# Autodesk Inventor assembly: drive
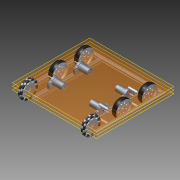
[picture p0: Inventor's stored thumbnail of the model, 180x180]
Saved by Autodesk Inventor 2013 (Build 170138000, 138)
## iProperties
Created: 2013-09-22
Part Number: drive
Document SubType Name: Assembly
Designer: Family Room
Mass: 858.54 g
Surface Area: 8628.43 cm^2
Volume: 788.69 cm^3
Density: 1.08856 g/cm^3
Author: Family Room
## Documents named in this file (12)
- C:\Users\cobrooks\Documents\GitHub\2013-2014_BlockParty\CAD\Drive\WIMP_mk2\drive.iam
- C:\Users\cobrooks\Documents\GitHub\2013-2014_BlockParty\CAD\Drive\Final Drive Complete\Frame Layer open.iam
- C:\Users\Family Room\Documents\Inventor\Content Center Files\R2011\en-US\ANSI B18.3(13)\ANSI B18.3 - 1_4-28 UNF - 1(22).ipt
- C:\Users\cobrooks\Documents\GitHub\2013-2014_BlockParty\CAD\Drive\Final Drive Complete\Tetrix Wheel 4 in omni.ipt
- C:\Users\cobrooks\Documents\GitHub\2013-2014_BlockParty\CAD\Drive\Final Drive Complete\Tetrix wheel 4 in.ipt
- C:\Users\cobrooks\Documents\GitHub\2013-2014_BlockParty\CAD\Drive\Final Drive Complete\pvc holder.ipt
- C:\Users\rihoobler\Documents\Inventor\tetrix_739091_2012.ipt
- U:\Imported Components\tetrix_739088_2012\tetrix_739088_2012.ipt
- U:\Imported Components\tetrix_739165_2012\tetrix_739165_2012.ipt
- U:\Imported Components\tetrix_739172_2012\tetrix_739172_2012.iam
- C:\Users\cobrooks\Documents\GitHub\2013-2014_BlockParty\CAD\Drive\Final Drive Complete\Motor Mount.ipt
- C:\Users\cobrooks\Documents\GitHub\2013-2014_BlockParty\CAD\Drive\Final Drive Complete\Motor.iam
## Components (61 placed, 11 different names)
1. Frame Layer open:1 [sub-assembly] — Insert:4, Insert:5, Insert:6, Mate:37, Mate:38, Flush:44, Mate:72, Flush:50, Mate:74, Flush:51, Mate:76, Flush:52, Flush:53, Mate:77, Flush:60
2. Spline Socket Head Cap Screw - Inch 1/4-28 UNF - 1:1
3. Spline Socket Head Cap Screw - Inch 1/4-28 UNF - 1:2
4. Spline Socket Head Cap Screw - Inch 1/4-28 UNF - 1:3
5. Spline Socket Head Cap Screw - Inch 1/4-28 UNF - 1:4 — Insert:4
6. Spline Socket Head Cap Screw - Inch 1/4-28 UNF - 1:5 — Insert:5
7. Spline Socket Head Cap Screw - Inch 1/4-28 UNF - 1:6 — Insert:6
8. Tetrix Wheel 4 in omni:1 — Mate:40, Mate:42, Mate:43, Flush:36, Insert:19
9. Tetrix Wheel 4 in omni:2 — Mate:41, Mate:44, Mate:45, Insert:24
10. Tetrix wheel 4 in:1 — Flush:34, Insert:26
11. Tetrix wheel 4 in:2 — Flush:34, Flush:35, Insert:25
12. Tetrix wheel 4 in:3 — Flush:36, Flush:37, Insert:21
13. Tetrix wheel 4 in:4 — Flush:37, Insert:22
14. pvc holder:1
15. pvc holder:2
16. pvc holder:3 — Mate:38
17. pvc holder:4 — Mate:37
18. Tetrix Wheel 4 in omni:3 — Mate:40, Mate:42, Mate:43, Insert:20
19. Tetrix Wheel 4 in omni:4 — Mate:41, Mate:44, Mate:45, Flush:35, Insert:27
20. tetrix_739091_2012:1 — Mate:50
21. tetrix_739091_2012:2 — Mate:61
22. tetrix_739091_2012:3
23. tetrix_739091_2012:4 — Mate:51
24. tetrix_739091_2012:5 — Mate:52
25. tetrix_739091_2012:6
26. tetrix_739091_2012:7
27. tetrix_739091_2012:8 — Flush:38, Mate:53
28. tetrix_739091_2012:9
29. tetrix_739091_2012:10 — Flush:38, Flush:39, Mate:54
30. tetrix_739091_2012:11
31. tetrix_739091_2012:12 — Flush:39, Mate:55, Mate:67
32. tetrix_739088_2012:1 — Mate:50
33. tetrix_739088_2012:2 — Mate:51, Flush:44, Flush:45, Mate:60
34. tetrix_739088_2012:3 — Mate:52, Flush:45, Mate:65
35. tetrix_739088_2012:4 — Mate:53
36. tetrix_739088_2012:5 — Mate:54, Mate:68, Mate:69
37. tetrix_739088_2012:6 — Mate:55, Mate:71
38. tetrix_739165_2012:1 — Insert:19, Flush:46
39. tetrix_739165_2012:2 — Mate:63, Mate:64, Mate:66, Flush:47
40. tetrix_739165_2012:3 — Mate:60, Flush:46, Mate:63, Mate:64, Insert:23
41. tetrix_739165_2012:4 — Mate:68, Flush:48, Insert:28
42. tetrix_739165_2012:5 — Insert:27, Flush:48
43. tetrix_739165_2012:6 — Mate:65, Flush:47
44. tetrix_739172_2012:1 [sub-assembly] — Insert:20, Mate:61
45. tetrix_739172_2012:2 [sub-assembly] — Insert:21
46. tetrix_739172_2012:3 [sub-assembly] — Insert:22
47. tetrix_739172_2012:4 [sub-assembly] — Insert:23, Mate:66
48. tetrix_739172_2012:5 [sub-assembly] — Insert:26, Mate:67
49. tetrix_739172_2012:6 [sub-assembly] — Insert:25
50. tetrix_739172_2012:7 [sub-assembly] — Insert:24
51. tetrix_739172_2012:8 [sub-assembly] — Insert:28, Mate:70
52. tetrix_739165_2012:7 — Mate:71, Flush:49
53. tetrix_739165_2012:8 — Mate:69, Mate:70, Flush:49
54. Motor Mount:1 — Mate:72, Flush:50, Flush:55, Mate:78, Flush:57
55. Motor Mount:2 — Mate:74, Flush:51, Flush:54, Mate:79, Flush:56
56. Motor Mount:3 — Mate:76, Flush:52, Flush:55, Mate:80, Flush:58
57. Motor Mount:4 — Flush:53, Mate:77, Flush:54, Mate:81, Flush:59
58. Motor:1 [sub-assembly] — Mate:78, Flush:57
59. Motor:2 [sub-assembly] — Mate:79, Flush:56
60. Motor:3 [sub-assembly] — Mate:80, Flush:58
61. Motor:4 [sub-assembly] — Mate:81, Flush:59
## Relationships (71: Mate 33, Flush 25, Insert 13)
- Insert:4: Frame Layer open:1 ↔ Spline Socket Head Cap Screw - Inch 1/4-28 UNF - 1:4
- Insert:5: Frame Layer open:1 ↔ Spline Socket Head Cap Screw - Inch 1/4-28 UNF - 1:5
- Insert:6: Frame Layer open:1 ↔ Spline Socket Head Cap Screw - Inch 1/4-28 UNF - 1:6
- Mate:37: Frame Layer open:1 ↔ pvc holder:4
- Mate:38: Frame Layer open:1 ↔ pvc holder:3
- Mate:40: Tetrix Wheel 4 in omni:1 ↔ Tetrix Wheel 4 in omni:3
- Mate:41: Tetrix Wheel 4 in omni:2 ↔ Tetrix Wheel 4 in omni:4
- Mate:42: Tetrix Wheel 4 in omni:1 ↔ Tetrix Wheel 4 in omni:3
- Mate:43: Tetrix Wheel 4 in omni:1 ↔ Tetrix Wheel 4 in omni:3
- Mate:44: Tetrix Wheel 4 in omni:2 ↔ Tetrix Wheel 4 in omni:4
- Mate:45: Tetrix Wheel 4 in omni:2 ↔ Tetrix Wheel 4 in omni:4
- Flush:34: Tetrix wheel 4 in:1 ↔ Tetrix wheel 4 in:2
- Flush:35: Tetrix wheel 4 in:2 ↔ Tetrix Wheel 4 in omni:4
- Flush:36: Tetrix Wheel 4 in omni:1 ↔ Tetrix wheel 4 in:3
- Flush:37: Tetrix wheel 4 in:3 ↔ Tetrix wheel 4 in:4
- Flush:38: tetrix_739091_2012:8 ↔ tetrix_739091_2012:10
- Flush:39: tetrix_739091_2012:10 ↔ tetrix_739091_2012:12
- Mate:50: tetrix_739091_2012:1 ↔ tetrix_739088_2012:1
- Mate:51: tetrix_739091_2012:4 ↔ tetrix_739088_2012:2
- Mate:52: tetrix_739091_2012:5 ↔ tetrix_739088_2012:3
- Mate:53: tetrix_739091_2012:8 ↔ tetrix_739088_2012:4
- Mate:54: tetrix_739091_2012:10 ↔ tetrix_739088_2012:5
- Mate:55: tetrix_739091_2012:12 ↔ tetrix_739088_2012:6
- Flush:44: Frame Layer open:1 ↔ tetrix_739088_2012:2
- Flush:45: tetrix_739088_2012:2 ↔ tetrix_739088_2012:3
- Insert:19: Tetrix Wheel 4 in omni:1 ↔ tetrix_739165_2012:1
- Mate:60: tetrix_739088_2012:2 ↔ tetrix_739165_2012:3
- Flush:46: tetrix_739165_2012:1 ↔ tetrix_739165_2012:3
- Insert:20: Tetrix Wheel 4 in omni:3 ↔ tetrix_739172_2012:1
- Mate:61: tetrix_739091_2012:2 ↔ tetrix_739172_2012:1
- Insert:21: Tetrix wheel 4 in:3 ↔ tetrix_739172_2012:2
- Insert:22: Tetrix wheel 4 in:4 ↔ tetrix_739172_2012:3
- Mate:63: tetrix_739165_2012:2 ↔ tetrix_739165_2012:3
- Mate:64: tetrix_739165_2012:2 ↔ tetrix_739165_2012:3
- Mate:65: tetrix_739088_2012:3 ↔ tetrix_739165_2012:6
- Insert:23: tetrix_739165_2012:3 ↔ tetrix_739172_2012:4
- Mate:66: tetrix_739165_2012:2 ↔ tetrix_739172_2012:4
- Flush:47: tetrix_739165_2012:2 ↔ tetrix_739165_2012:6
- Insert:24: Tetrix Wheel 4 in omni:2 ↔ tetrix_739172_2012:7
- Insert:25: Tetrix wheel 4 in:2 ↔ tetrix_739172_2012:6
- Insert:26: Tetrix wheel 4 in:1 ↔ tetrix_739172_2012:5
- Mate:67: tetrix_739091_2012:12 ↔ tetrix_739172_2012:5
- Insert:27: Tetrix Wheel 4 in omni:4 ↔ tetrix_739165_2012:5
- Mate:68: tetrix_739088_2012:5 ↔ tetrix_739165_2012:4
- Flush:48: tetrix_739165_2012:4 ↔ tetrix_739165_2012:5
- Insert:28: tetrix_739165_2012:4 ↔ tetrix_739172_2012:8
- Mate:69: tetrix_739088_2012:5 ↔ tetrix_739165_2012:8
- Mate:70: tetrix_739172_2012:8 ↔ tetrix_739165_2012:8
- Mate:71: tetrix_739088_2012:6 ↔ tetrix_739165_2012:7
- Flush:49: tetrix_739165_2012:7 ↔ tetrix_739165_2012:8
- Mate:72: Frame Layer open:1 ↔ Motor Mount:1
- Flush:50: Frame Layer open:1 ↔ Motor Mount:1
- Mate:74: Frame Layer open:1 ↔ Motor Mount:2
- Flush:51: Frame Layer open:1 ↔ Motor Mount:2
- Mate:76: Frame Layer open:1 ↔ Motor Mount:3
- Flush:52: Frame Layer open:1 ↔ Motor Mount:3
- Flush:53: Frame Layer open:1 ↔ Motor Mount:4
- Mate:77: Frame Layer open:1 ↔ Motor Mount:4
- Flush:54: Motor Mount:2 ↔ Motor Mount:4
- Flush:55: Motor Mount:1 ↔ Motor Mount:3
- Mate:78: Motor Mount:1 ↔ Motor:1
- Mate:79: Motor Mount:2 ↔ Motor:2
- Mate:80: Motor Mount:3 ↔ Motor:3
- Mate:81: Motor Mount:4 ↔ Motor:4
- Flush:56: Motor Mount:2 ↔ Motor:2
- Flush:57: Motor Mount:1 ↔ Motor:1
- Flush:58: Motor Mount:3 ↔ Motor:3
- Flush:59: Motor Mount:4 ↔ Motor:4
- Flush:60 (12.7 mm): Frame Layer open:1
- Flush:61 (17.907 mm)
- Flush:62 (-17.907 mm)
